# Autodesk Inventor assembly: Support Structure
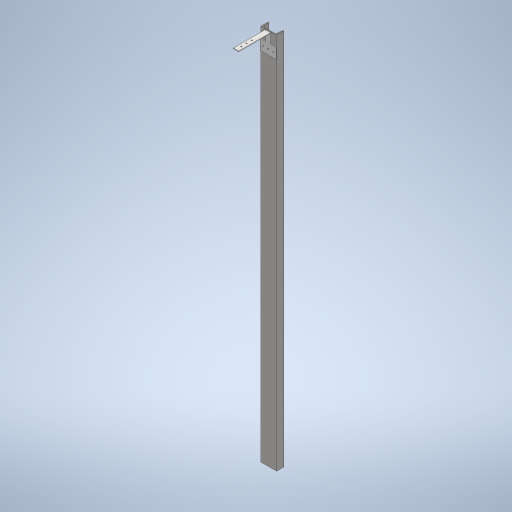
[picture p0: Inventor's stored thumbnail of the model, 512x512]
Saved by Autodesk Inventor 2023 (Build 270158000, 158)
## iProperties
RuleStatus: InUse
Created: 2022-07-19
Part Number: Support Structure
Document SubType Name: Assembly
Designer: EricPaul
Author: EricPaul
## Documents named in this file (4)
- C:\Users\EricPaul\Documents\AVA\202207 Model States\Support Structure.iam
- C:\Users\EricPaul\Documents\AVA\202207 Model States\AISC - C 3 x 3.5 - 72.ipt
- C:\Users\EricPaul\Documents\AVA\202207 Model States\Flexible Bracket.ipt
- C:\Users\EricPaul\Documents\AVA\202207 Model States\Top Brace.ipt
## Components (15 placed, 15 different names)
1. C Channel 1 Right — Flush:1, Flush:2, Flush:3, Flush:4, Mate:1, Mate:7
2. Flexible Bracket 1 Right — Flush:3, Flush:4, Mate:1
3. C Channel 1 Left — Flush:17, Flush:20, Flush:23
4. Flexible Bracket 1 Left
5. Top Brace 1 — Mate:14, Flush:26, Flush:27
6. C Channel 2 Right — Mate:8, Mate:10, Flush:15, Mate:12, Mate:17
7. Flexible Bracket 2 Right
8. C Channel 2 Left — Flush:18, Flush:21, Mate:12
9. Flexible Bracket 2 Left
10. Top Brace 2 — Mate:15, Flush:25, Mate:17
11. C Channel 3 Right — Mate:9, Mate:11, Flush:16, Mate:13, Mate:18
12. Flexible Bracket 3 Right
13. C Channel 3 Left — Flush:19, Flush:22, Mate:13
14. Flexible Bracket 3 Left
15. Top Brace 3 — Mate:16, Flush:24, Mate:18
## Relationships (45: Flush 27, Mate 18)
- Flush:1: C Channel 1 Right
- Flush:2: C Channel 1 Right
- Flush:3: C Channel 1 Right ↔ Flexible Bracket 1 Right
- Flush:4: C Channel 1 Right ↔ Flexible Bracket 1 Right
- Mate:1 (-100.8016 mm): C Channel 1 Right ↔ Flexible Bracket 1 Right
- [Flush]: C Channel 2 Right ↔ Flexible Bracket 2 Right
- [Flush]: C Channel 2 Right ↔ Flexible Bracket 2 Right
- [Mate] (-100.8016 mm): C Channel 2 Right ↔ Flexible Bracket 2 Right
- [Flush]: C Channel 3 Right ↔ Flexible Bracket 3 Right
- [Flush]: C Channel 3 Right ↔ Flexible Bracket 3 Right
- [Mate] (-100.8016 mm): C Channel 3 Right ↔ Flexible Bracket 3 Right
- [Flush]: C Channel 1 Left ↔ Flexible Bracket 1 Left
- [Flush]: C Channel 1 Left ↔ Flexible Bracket 1 Left
- [Mate] (-100.8016 mm): C Channel 1 Left ↔ Flexible Bracket 1 Left
- [Flush]: C Channel 2 Left ↔ Flexible Bracket 2 Left
- [Flush]: C Channel 2 Left ↔ Flexible Bracket 2 Left
- [Mate] (-100.8016 mm): C Channel 2 Left ↔ Flexible Bracket 2 Left
- [Flush]: C Channel 3 Left ↔ Flexible Bracket 3 Left
- [Flush]: C Channel 3 Left ↔ Flexible Bracket 3 Left
- [Mate] (-100.8016 mm): C Channel 3 Left ↔ Flexible Bracket 3 Left
- Mate:7: C Channel 1 Right
- Mate:8: C Channel 2 Right
- Mate:9: C Channel 3 Right
- Mate:10 (-381 mm): C Channel 2 Right
- Mate:11 (-762 mm): C Channel 3 Right
- Flush:15: C Channel 2 Right
- Flush:16: C Channel 3 Right
- Flush:17: C Channel 1 Left
- Flush:18: C Channel 2 Left
- Flush:19: C Channel 3 Left
- Flush:20 (-1016 mm): C Channel 1 Left
- Flush:21 (-1016 mm): C Channel 2 Left
- Flush:22 (-1016 mm): C Channel 3 Left
- Flush:23: C Channel 1 Left
- Mate:12: C Channel 2 Right ↔ C Channel 2 Left
- Mate:13: C Channel 3 Right ↔ C Channel 3 Left
- Mate:14: Top Brace 1
- Mate:15: Top Brace 2
- Mate:16: Top Brace 3
- Flush:24 (1879.6 mm): Top Brace 3
- Flush:25 (-1854.2 mm): Top Brace 2
- Flush:26 (1828.8 mm): Top Brace 1
- Flush:27: Top Brace 1
- Mate:17: C Channel 2 Right ↔ Top Brace 2
- Mate:18: C Channel 3 Right ↔ Top Brace 3
## Named parameters: Support1Distance = 76.2 mm, d8_d3 = 0 mm, d9_d6 = 0 mm, d10_d7 = -100.80159 mm, d11_d3 = 0 mm, d12_d6 = 0 mm, d13_d7 = -100.80159 mm, d14_d3 = 0 mm, d15_d6 = 0 mm, d16_d7 = -100.80159 mm, d17_d3 = 0 mm, d18_d6 = 0 mm, d19_d7 = -100.80159 mm, d20_d3 = 0 mm, d21_d6 = 0 mm, d22_d7 = -100.80159 mm, Support2Distance = 101.6 mm, Support3Distance = 127 mm
